# Autodesk Inventor assembly: 2x3pins
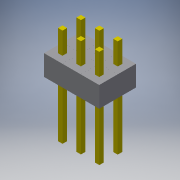
[picture p0: Inventor's stored thumbnail of the model, 180x180]
Saved by Autodesk Inventor 2019 (Build 230136000, 136)
## iProperties
Created: 2019-07-16
Part Number: 2x3pins
Document SubType Name: Assembly
Designer: james
Author: james
## Documents named in this file (2)
- F:\JimsDesign\P1001-16bit-CPU\P1001-001 - 16bit CPU\P1001-001-210 - CAD Library\2x3pins.iam
- F:\JimsDesign\P1001-16bit-CPU\P1001-001 - 16bit CPU\P1001-001-210 - CAD Library\1x2Pins.iam
## Components (3 placed, 1 different names)
1. 1x2Pins:1 [sub-assembly] — Mate:2, Flush:1, Flush:3
2. 1x2Pins:2 [sub-assembly] — Mate:1, Mate:2, Flush:1, Flush:2, Flush:3, Flush:4
3. 1x2Pins:3 [sub-assembly] — Mate:1, Flush:2, Flush:4
## Relationships (6: Flush 4, Mate 2)
- Mate:1: 1x2Pins:2 ↔ 1x2Pins:3
- Mate:2: 1x2Pins:1 ↔ 1x2Pins:2
- Flush:1: 1x2Pins:1 ↔ 1x2Pins:2
- Flush:2: 1x2Pins:2 ↔ 1x2Pins:3
- Flush:3: 1x2Pins:1 ↔ 1x2Pins:2
- Flush:4: 1x2Pins:2 ↔ 1x2Pins:3
